# Autodesk Inventor assembly: EXCISS
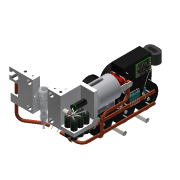
[picture p0: Inventor's stored thumbnail of the model, 180x180]
Saved by Autodesk Inventor 2017 (Build 210142000, 142)
## iProperties
Part Number: EXCISS
Material: Generisch
Document SubType Name: Assembly
Designer: Philomena-Theresa
Author: Philomena-Theresa
## Documents named in this file (28)
- C:\Seafile\Meine Bibliothek\Inventor\EXCISS\2019\HVU\HVU.iam
- C:\Seafile\Meine Bibliothek\Inventor\EXCISS\2019\HVU\HVU_sample_chamber_mount_plus.ipt
- C:\Seafile\Meine Bibliothek\Inventor\EXCISS\2019\HVU\HVU_PTFE_sleeve.ipt
- C:\Seafile\Meine Bibliothek\Inventor\EXCISS\2019\HVU\HVU_1N4007.ipt
- C:\Seafile\Meine Bibliothek\Inventor\EXCISS\2019\HVU\HVU_thyristor(TN2540-800G-TR).ipt
- C:\Seafile\Meine Bibliothek\Inventor\EXCISS\2019\HVU\HVU_ignition_coil.ipt
- C:\Seafile\Meine Bibliothek\Inventor\EXCISS\2019\HVU\HVU_DC_DC_converter_(M1730CQEA06065).ipt
- C:\Seafile\Meine Bibliothek\Inventor\EXCISS\2019\HVU\HVU_capacitor_MKP4_0,1µF_(450377).ipt
- C:\Seafile\Meine Bibliothek\Inventor\EXCISS\2019\HVU\HVU_capacitor_150µF_(LGN2X151MELB50).ipt
- C:\Seafile\Meine Bibliothek\Inventor\EXCISS\2019\HVU\HVU_resistor_WHS7_68R.ipt
- C:\Seafile\Meine Bibliothek\Inventor\EXCISS\2019\HVU\HVU_schunt.ipt
- C:\Seafile\Meine Bibliothek\Inventor\EXCISS\2019\HVU\HVU_PCB_trigger.ipt
- C:\Seafile\Meine Bibliothek\Inventor\EXCISS\2019\HVU\HVU_PCB_power_switch.ipt
- C:\Seafile\Meine Bibliothek\Inventor\EXCISS\2019\HVU\HVU_ferrit_cable_core_(28B0773-050).ipt
- C:\Seafile\Meine Bibliothek\Inventor\EXCISS\2019\HVU\HVU_sample_chamber_mount_minus.ipt
- C:\Seafile\Meine Bibliothek\Inventor\EXCISS\2019\HVU\HVU_sample_chamber.iam
- C:\Seafile\Meine Bibliothek\Inventor\EXCISS\2019\HVU\HVU_resistor_1M5_(VR25000001504JA100).ipt
- C:\Seafile\Meine Bibliothek\Inventor\EXCISS\2019\HVU\HVU_resistor_5M1_(VR25000005104JA100).ipt
- C:\Seafile\Meine Bibliothek\Inventor\EXCISS\2019\HVU\HVU_resistor_2M2_(VR25000002204JA100).ipt
- C:\Seafile\Meine Bibliothek\Inventor\EXCISS\2019\HVU\HVU_wires_Darc.ipt
- C:\Seafile\Meine Bibliothek\Inventor\EXCISS\2019\HVU\HVU_ignition_coil_stud.ipt
- C:\Seafile\Meine Bibliothek\Inventor\EXCISS\2019\HVU\HVU_wires_Carc.ipt
- C:\Seafile\Meine Bibliothek\Inventor\EXCISS\2019\HVU\HVU_wires_resistor_WHS7.ipt
- C:\Seafile\Meine Bibliothek\Inventor\EXCISS\2019\HVU\HVU_wires_resistor.ipt
- C:\Seafile\Meine Bibliothek\Inventor\EXCISS\2019\HVU\HVU_wires_diodes.ipt
- C:\Seafile\Meine Bibliothek\Inventor\EXCISS\2019\HVU\HVU_diode_(BY16).ipt
- C:\Seafile\Meine Bibliothek\Inventor\EXCISS\2019\HVU\HVU_DIN_934_M3x0,5.ipt
- C:\Seafile\Meine Bibliothek\Inventor\EXCISS\2019\HVU\HVU_standoff_(DA_40MM).ipt
## Components (49 placed, 27 different names)
1. HVU_sample_chamber_mount_plus:1 — Passend:28, Fluchtend:6, Passend:47, Fluchtend:13, Passend:48, Passend:49, Passend:50, Passend:51, Passend:53, Passend:54, Passend:58, Winkel:3, Fluchtend:25, Passend:94, Fluchtend:27, Passend:102, Passend:103, Passend:104, Fluchtend:36, Fluchtend:39, Passend:117, Passend:118, Fluchtend:46, Fluchtend:52, Passend:147, Passend:152, Winkel:12, Winkel:13
2. HVU_PTFE_sleeve:1 — Passend:28, Fluchtend:6, Passend:92
3. HVU_1N4007:1 — Passend:34, Passend:36, Passend:171, Passend:173, Fluchtend:89, Fluchtend:90
4. HVU_thyristor(TN2540-800G-TR):1 — Passend:34, Passend:36, Passend:37, Winkel:2, Passend:39, Fluchtend:9, Fluchtend:79, Passend:171
5. HVU_ignition_coil:1 — Passend:37, Winkel:2, Passend:58, Winkel:3, Passend:123, Fluchtend:50, Fluchtend:51, Fluchtend:80, Passend:169, Fluchtend:88
6. HVU_DC_DC_converter_(M1730CQEA06065):1 — Passend:79, Fluchtend:43, Passend:149, Winkel:11, Passend:160, Passend:161, Passend:162, Passend:163, Passend:164, Passend:165, Fluchtend:91, Fluchtend:92, Fluchtend:93, Fluchtend:95, Fluchtend:96, Passend:175, Passend:176, Passend:177
7. HVU_capacitor_MKP4_0,1µF_(450377):1 — Passend:39, Fluchtend:9, Passend:56, Fluchtend:22, Passend:161, Passend:167, Passend:168, Fluchtend:78, Fluchtend:79, Fluchtend:80, Passend:169, Fluchtend:81, Passend:170, Fluchtend:83, Fluchtend:85, Passend:174
8. HVU_resistor_2M2_(VR25000002204JA100):1 — Passend:167, Passend:168, Fluchtend:78, Passend:172, Fluchtend:86, Fluchtend:87
9. HVU_diode_(BY16):1 — Passend:47, Fluchtend:13, Passend:101, Fluchtend:34, Fluchtend:35, Passend:123
10. HVU_diode_(BY16):2 — Passend:49, Passend:78, Fluchtend:27, Fluchtend:28, Fluchtend:29, Fluchtend:30, Fluchtend:31, Fluchtend:32, Passend:95, Passend:100
11. HVU_diode_(BY16):3 — Passend:48, Fluchtend:28, Passend:95
12. HVU_diode_(BY16):4 — Passend:53, Passend:77, Fluchtend:31, Passend:96, Passend:98, Passend:111, Fluchtend:45
13. HVU_diode_(BY16):5 — Passend:54, Fluchtend:32, Passend:96, Fluchtend:33, Passend:112
14. HVU_diode_(BY16):6 — Passend:51, Passend:77, Passend:78, Fluchtend:30, Passend:97, Passend:99
15. HVU_diode_(BY16):7 — Passend:50, Fluchtend:29, Passend:97
16. HVU_1N4007:2 — Passend:56, Fluchtend:22, Passend:170, Fluchtend:82, Fluchtend:84
17. HVU_resistor_5M1_(VR25000005104JA100):1 — Passend:155, Fluchtend:66, Passend:158, Fluchtend:72
18. HVU_1N4007:3 — Passend:144, Passend:145, Passend:152, Passend:166, Fluchtend:74, Fluchtend:75, Fluchtend:77
19. HVU_thyristor(TN2540-800G-TR):2 — Passend:144, Passend:145, Passend:150, Passend:151, Passend:153, Passend:166, Fluchtend:76
20. HVU_resistor_WHS7_68R:2 — Passend:72, Fluchtend:58, Passend:147, Passend:148, Passend:149
21. HVU_resistor_WHS7_68R:3 — Passend:72, Fluchtend:53, Fluchtend:58, Passend:148, Passend:150, Passend:153, Fluchtend:61, Fluchtend:62, Fluchtend:63, Fluchtend:64, Fluchtend:65
22. HVU_schunt:1 — Fluchtend:47, Passend:137, Passend:138, Passend:139
23. HVU_PCB_trigger:1 — Passend:79, Winkel:11, Passend:164, Fluchtend:99
24. HVU_PCB_power_switch:1 — Passend:177, Fluchtend:100, Passend:178
25. HVU_ferrit_cable_core_(28B0773-050):1 — Passend:175, Passend:176, Fluchtend:99, Fluchtend:100, Passend:178
26. HVU_sample_chamber_mount_minus:1 — Passend:93, Fluchtend:25, Passend:94, Winkel:7, Passend:113, Passend:114, Fluchtend:48, Fluchtend:49
27. HVU_sample_chamber:1 [sub-assembly] — Passend:92, Passend:93, Winkel:7
28. HVU_ignition_coil_stud:1 — Passend:103, Fluchtend:37
29. HVU_ignition_coil_stud:2 — Passend:102, Fluchtend:36, Fluchtend:37, Fluchtend:38
30. HVU_ignition_coil_stud:3 — Passend:104, Fluchtend:38
31. HVU_wires_Carc:1 — Fluchtend:40, Passend:105, Passend:106, Passend:107, Passend:108, Passend:109, Passend:110, Passend:111, Passend:112, Passend:132, Passend:133, Winkel:9, Fluchtend:48, Fluchtend:49, Fluchtend:50, Fluchtend:51, Fluchtend:52
32. HVU_wires_Darc:1 — Fluchtend:33, Passend:98, Passend:99, Passend:100, Passend:101, Fluchtend:34, Fluchtend:35, Fluchtend:45, Passend:132, Passend:133
33. HVU_wires_resistor_WHS7:1 — Fluchtend:60, Fluchtend:61, Fluchtend:62, Fluchtend:63, Fluchtend:64, Fluchtend:65
34. HVU_wires_resistor:1 — Fluchtend:68, Fluchtend:69, Fluchtend:70, Fluchtend:71, Fluchtend:72, Fluchtend:73, Passend:172, Fluchtend:85, Fluchtend:86, Fluchtend:87, Fluchtend:91, Fluchtend:94, Fluchtend:95, Fluchtend:96, Fluchtend:97, Fluchtend:98
35. HVU_wires_diodes:1 — Fluchtend:75, Fluchtend:76, Fluchtend:77, Fluchtend:81, Fluchtend:82, Fluchtend:83, Fluchtend:84, Passend:173, Fluchtend:88, Fluchtend:89, Fluchtend:90
36. HVU_resistor_1M5_(VR25000001504JA100):7 — Fluchtend:92, Fluchtend:93, Fluchtend:94, Passend:174, Fluchtend:97, Fluchtend:98
37. DIN 934 - ersetzt durch DIN EN 24032/28673/28674 M3:3 — Passend:181, Winkel:14
38. DIN 934 - ersetzt durch DIN EN 24032/28673/28674 M3:4 — Passend:182, Winkel:14
39. HVU_resistor_1M5_(VR25000001504JA100):1 — Passend:155, Fluchtend:66, Passend:158, Passend:162, Fluchtend:67, Fluchtend:69, Passend:165, Fluchtend:71
40. HVU_resistor_1M5_(VR25000001504JA100):2 — Fluchtend:70
41. HVU_resistor_1M5_(VR25000001504JA100):3
42. HVU_resistor_1M5_(VR25000001504JA100):4
43. HVU_resistor_1M5_(VR25000001504JA100):5
44. HVU_resistor_1M5_(VR25000001504JA100):6 — Passend:163, Fluchtend:73
45. HVU_capacitor_150µF_(LGN2X151MELB50):1 — Passend:107, Passend:110, Passend:126, Passend:179, Fluchtend:101
46. HVU_capacitor_150µF_(LGN2X151MELB50):2 — Passend:106, Passend:109, Passend:180
47. HVU_capacitor_150µF_(LGN2X151MELB50):3 — Passend:105, Passend:108, Passend:124, Passend:125, Passend:139, Winkel:12
48. HVU_standoff_(DA_40MM):1 — Passend:179, Passend:180, Winkel:13, Fluchtend:101, Passend:181
49. HVU_standoff_(DA_40MM):2 — Passend:182
## Component patterns: (6 elements, first: HVU_resistor_1M5_(VR25000001504JA100):1), (3 elements, first: HVU_capacitor_150µF_(LGN2X151MELB50):1), (2 elements, first: HVU_standoff_(DA_40MM):1)
## Relationships (183: Mate 98, Flush 75, Angle 9, Symmetry 1)
- Passend:28 [Mate]: HVU_sample_chamber_mount_plus:1 ↔ HVU_PTFE_sleeve:1
- Fluchtend:6 [Flush] (-5.67 mm): HVU_sample_chamber_mount_plus:1 ↔ HVU_PTFE_sleeve:1
- Passend:34 [Mate] (0.39 mm): HVU_1N4007:1 ↔ HVU_thyristor(TN2540-800G-TR):1
- Passend:36 [Mate]: HVU_1N4007:1 ↔ HVU_thyristor(TN2540-800G-TR):1
- Passend:37 [Mate]: HVU_thyristor(TN2540-800G-TR):1 ↔ HVU_ignition_coil:1
- Winkel:2 [Angle] (0 deg): HVU_thyristor(TN2540-800G-TR):1 ↔ HVU_ignition_coil:1
- Passend:39 [Mate]: HVU_thyristor(TN2540-800G-TR):1 ↔ HVU_capacitor_MKP4_0,1µF_(450377):1
- Fluchtend:9 [Flush]: HVU_thyristor(TN2540-800G-TR):1 ↔ HVU_capacitor_MKP4_0,1µF_(450377):1
- Passend:47 [Mate]: HVU_sample_chamber_mount_plus:1 ↔ HVU_diode_(BY16):1
- Fluchtend:13 [Flush] (-1 mm): HVU_sample_chamber_mount_plus:1 ↔ HVU_diode_(BY16):1
- Passend:48 [Mate]: HVU_sample_chamber_mount_plus:1 ↔ HVU_diode_(BY16):3
- Passend:49 [Mate]: HVU_sample_chamber_mount_plus:1 ↔ HVU_diode_(BY16):2
- Passend:50 [Mate]: HVU_sample_chamber_mount_plus:1 ↔ HVU_diode_(BY16):7
- Passend:51 [Mate]: HVU_sample_chamber_mount_plus:1 ↔ HVU_diode_(BY16):6
- Passend:53 [Mate]: HVU_sample_chamber_mount_plus:1 ↔ HVU_diode_(BY16):4
- Passend:54 [Mate]: HVU_sample_chamber_mount_plus:1 ↔ HVU_diode_(BY16):5
- Passend:56 [Mate] (1.5 mm): HVU_capacitor_MKP4_0,1µF_(450377):1 ↔ HVU_1N4007:2
- Fluchtend:22 [Flush]: HVU_capacitor_MKP4_0,1µF_(450377):1 ↔ HVU_1N4007:2
- Passend:58 [Mate] (3 mm): HVU_sample_chamber_mount_plus:1 ↔ HVU_ignition_coil:1
- Winkel:3 [Angle] (270 deg): HVU_sample_chamber_mount_plus:1 ↔ HVU_ignition_coil:1
- Passend:72 [Mate] (9 mm): HVU_resistor_WHS7_68R:2 ↔ HVU_resistor_WHS7_68R:3
- Passend:77 [Mate]: HVU_diode_(BY16):4 ↔ HVU_diode_(BY16):6
- Passend:78 [Mate]: HVU_diode_(BY16):2 ↔ HVU_diode_(BY16):6
- Passend:79 [Mate] (1 mm): HVU_DC_DC_converter_(M1730CQEA06065):1 ↔ HVU_PCB_trigger:1
- Passend:92 [Mate]: HVU_PTFE_sleeve:1 ↔ HVU_sample_chamber:1
- Passend:93 [Mate]: HVU_sample_chamber_mount_minus:1 ↔ HVU_sample_chamber:1
- Fluchtend:25 [Flush]: HVU_sample_chamber_mount_plus:1 ↔ HVU_sample_chamber_mount_minus:1
- Passend:94 [Mate] (30 mm): HVU_sample_chamber_mount_plus:1 ↔ HVU_sample_chamber_mount_minus:1
- Winkel:7 [Angle] (0 deg): HVU_sample_chamber_mount_minus:1 ↔ HVU_sample_chamber:1
- Fluchtend:27 [Flush] (6 mm): HVU_sample_chamber_mount_plus:1 ↔ HVU_diode_(BY16):2
- Fluchtend:28 [Flush]: HVU_diode_(BY16):2 ↔ HVU_diode_(BY16):3
- Fluchtend:29 [Flush]: HVU_diode_(BY16):2 ↔ HVU_diode_(BY16):7
- Fluchtend:30 [Flush]: HVU_diode_(BY16):2 ↔ HVU_diode_(BY16):6
- Fluchtend:31 [Flush]: HVU_diode_(BY16):2 ↔ HVU_diode_(BY16):4
- Fluchtend:32 [Flush]: HVU_diode_(BY16):2 ↔ HVU_diode_(BY16):5
- Passend:95 [Mate]: HVU_diode_(BY16):2 ↔ HVU_diode_(BY16):3
- Passend:96 [Mate]: HVU_diode_(BY16):4 ↔ HVU_diode_(BY16):5
- Passend:97 [Mate]: HVU_diode_(BY16):6 ↔ HVU_diode_(BY16):7
- Fluchtend:33 [Flush]: HVU_diode_(BY16):5 ↔ HVU_wires_Darc:1
- Passend:98 [Mate]: HVU_diode_(BY16):4 ↔ HVU_wires_Darc:1
- Passend:99 [Mate]: HVU_diode_(BY16):6 ↔ HVU_wires_Darc:1
- Passend:100 [Mate]: HVU_diode_(BY16):2 ↔ HVU_wires_Darc:1
- Passend:101 [Mate]: HVU_diode_(BY16):1 ↔ HVU_wires_Darc:1
- Fluchtend:34 [Flush]: HVU_diode_(BY16):1 ↔ HVU_wires_Darc:1
- Fluchtend:35 [Flush]: HVU_diode_(BY16):1 ↔ HVU_wires_Darc:1
- Passend:102 [Mate]: HVU_sample_chamber_mount_plus:1 ↔ HVU_ignition_coil_stud:2
- Passend:103 [Mate]: HVU_sample_chamber_mount_plus:1 ↔ HVU_ignition_coil_stud:1
- Passend:104 [Mate]: HVU_sample_chamber_mount_plus:1 ↔ HVU_ignition_coil_stud:3
- Fluchtend:36 [Flush]: HVU_sample_chamber_mount_plus:1 ↔ HVU_ignition_coil_stud:2
- Fluchtend:37 [Flush]: HVU_ignition_coil_stud:1 ↔ HVU_ignition_coil_stud:2
- Fluchtend:38 [Flush]: HVU_ignition_coil_stud:2 ↔ HVU_ignition_coil_stud:3
- Fluchtend:39 [Flush] (-9 mm): HVU_sample_chamber_mount_plus:1
- Fluchtend:40 [Flush]: HVU_wires_Carc:1
- Passend:105 [Mate]: HVU_wires_Carc:1 ↔ HVU_capacitor_150µF_(LGN2X151MELB50):3
- Passend:106 [Mate]: HVU_wires_Carc:1 ↔ HVU_capacitor_150µF_(LGN2X151MELB50):2
- Passend:107 [Mate]: HVU_wires_Carc:1 ↔ HVU_capacitor_150µF_(LGN2X151MELB50):1
- Passend:108 [Mate]: HVU_wires_Carc:1 ↔ HVU_capacitor_150µF_(LGN2X151MELB50):3
- Passend:109 [Mate]: HVU_wires_Carc:1 ↔ HVU_capacitor_150µF_(LGN2X151MELB50):2
- Passend:110 [Mate]: HVU_wires_Carc:1 ↔ HVU_capacitor_150µF_(LGN2X151MELB50):1
- Passend:111 [Mate]: HVU_diode_(BY16):4 ↔ HVU_wires_Carc:1
- Passend:112 [Mate]: HVU_diode_(BY16):5 ↔ HVU_wires_Carc:1
- Passend:113 [Mate]: HVU_sample_chamber_mount_minus:1
- Passend:114 [Mate]: HVU_sample_chamber_mount_minus:1
- Passend:115 [Mate]
- Passend:116 [Mate]
- Passend:117 [Mate]: HVU_sample_chamber_mount_plus:1
- Passend:118 [Mate]: HVU_sample_chamber_mount_plus:1
- Passend:119 [Mate]
- Passend:120 [Mate]
- Fluchtend:41 [Flush] (-5 mm)
- Fluchtend:42 [Flush] (-5 mm)
- Fluchtend:43 [Flush] (0.4 mm): HVU_DC_DC_converter_(M1730CQEA06065):1
- Passend:121 [Mate]
- Passend:122 [Mate]
- Fluchtend:44 [Flush] (-5 mm)
- Passend:123 [Mate]: HVU_ignition_coil:1 ↔ HVU_diode_(BY16):1
- Passend:124 [Mate] (2.125 mm): HVU_capacitor_150µF_(LGN2X151MELB50):3
- Passend:125 [Mate]: HVU_capacitor_150µF_(LGN2X151MELB50):3
- Passend:126 [Mate]: HVU_capacitor_150µF_(LGN2X151MELB50):1
- Passend:127 [Mate]
- Passend:128 [Mate]
- Passend:129 [Mate] (-15.5 mm)
- Fluchtend:45 [Flush]: HVU_diode_(BY16):4 ↔ HVU_wires_Darc:1
- Passend:132 [Mate]: HVU_wires_Carc:1 ↔ HVU_wires_Darc:1
- Passend:133 [Mate]: HVU_wires_Carc:1 ↔ HVU_wires_Darc:1
- Fluchtend:46 [Flush] (7 mm): HVU_sample_chamber_mount_plus:1
- Passend:134 [Mate]
- Passend:135 [Mate]
- Passend:136 [Mate]
- Winkel:8 [Angle] (45 deg)
- Fluchtend:47 [Flush] (0.5 mm): HVU_schunt:1
- Symmetrie:1
- Passend:137 [Mate]: HVU_schunt:1
- Winkel:9 [Angle] (90 deg): HVU_wires_Carc:1
- Passend:138 [Mate] (5.5 mm): HVU_schunt:1
- Passend:139 [Mate] (15.5 mm): HVU_schunt:1 ↔ HVU_capacitor_150µF_(LGN2X151MELB50):3
- Fluchtend:48 [Flush]: HVU_sample_chamber_mount_minus:1 ↔ HVU_wires_Carc:1
- Fluchtend:49 [Flush]: HVU_sample_chamber_mount_minus:1 ↔ HVU_wires_Carc:1
- Fluchtend:50 [Flush]: HVU_ignition_coil:1 ↔ HVU_wires_Carc:1
- Fluchtend:51 [Flush]: HVU_ignition_coil:1 ↔ HVU_wires_Carc:1
- Fluchtend:52 [Flush]: HVU_sample_chamber_mount_plus:1 ↔ HVU_wires_Carc:1
- Fluchtend:53 [Flush]: HVU_resistor_WHS7_68R:3
- Fluchtend:58 [Flush]: HVU_resistor_WHS7_68R:2 ↔ HVU_resistor_WHS7_68R:3
- Passend:144 [Mate] (0.39 mm): HVU_1N4007:3 ↔ HVU_thyristor(TN2540-800G-TR):2
- Passend:145 [Mate] (-1.2 mm): HVU_1N4007:3 ↔ HVU_thyristor(TN2540-800G-TR):2
- Passend:147 [Mate] (-4.6 mm): HVU_sample_chamber_mount_plus:1 ↔ HVU_resistor_WHS7_68R:2
- Passend:148 [Mate]: HVU_resistor_WHS7_68R:2 ↔ HVU_resistor_WHS7_68R:3
- Passend:149 [Mate] (-4.5 mm): HVU_DC_DC_converter_(M1730CQEA06065):1 ↔ HVU_resistor_WHS7_68R:2
- Passend:150 [Mate] (3 mm): HVU_thyristor(TN2540-800G-TR):2 ↔ HVU_resistor_WHS7_68R:3
- Passend:151 [Mate] (-1 mm): HVU_thyristor(TN2540-800G-TR):2
- Passend:152 [Mate] (35.5 mm): HVU_sample_chamber_mount_plus:1 ↔ HVU_1N4007:3
- Passend:153 [Mate] (-2 mm): HVU_thyristor(TN2540-800G-TR):2 ↔ HVU_resistor_WHS7_68R:3
- Fluchtend:60 [Flush]: HVU_wires_resistor_WHS7:1
- Fluchtend:61 [Flush]: HVU_resistor_WHS7_68R:3 ↔ HVU_wires_resistor_WHS7:1
- Fluchtend:62 [Flush]: HVU_resistor_WHS7_68R:3 ↔ HVU_wires_resistor_WHS7:1
- Fluchtend:63 [Flush]: HVU_resistor_WHS7_68R:3 ↔ HVU_wires_resistor_WHS7:1
- Fluchtend:64 [Flush]: HVU_resistor_WHS7_68R:3 ↔ HVU_wires_resistor_WHS7:1
- Fluchtend:65 [Flush]: HVU_resistor_WHS7_68R:3 ↔ HVU_wires_resistor_WHS7:1
- Passend:155 [Mate]: HVU_resistor_5M1_(VR25000005104JA100):1 ↔ HVU_resistor_1M5_(VR25000001504JA100):1
- Fluchtend:66 [Flush]: HVU_resistor_5M1_(VR25000005104JA100):1 ↔ HVU_resistor_1M5_(VR25000001504JA100):1
- Passend:158 [Mate] (8 mm): HVU_resistor_5M1_(VR25000005104JA100):1 ↔ HVU_resistor_1M5_(VR25000001504JA100):1
- Winkel:11 [Angle] (0 deg): HVU_DC_DC_converter_(M1730CQEA06065):1 ↔ HVU_PCB_trigger:1
- Passend:160 [Mate]: HVU_DC_DC_converter_(M1730CQEA06065):1
- Passend:161 [Mate] (1 mm): HVU_DC_DC_converter_(M1730CQEA06065):1 ↔ HVU_capacitor_MKP4_0,1µF_(450377):1
- Passend:162 [Mate] (-0.5 mm): HVU_DC_DC_converter_(M1730CQEA06065):1 ↔ HVU_resistor_1M5_(VR25000001504JA100):1
- Passend:163 [Mate] (4 mm): HVU_DC_DC_converter_(M1730CQEA06065):1 ↔ HVU_resistor_1M5_(VR25000001504JA100):6
- Passend:164 [Mate]: HVU_DC_DC_converter_(M1730CQEA06065):1 ↔ HVU_PCB_trigger:1
- Fluchtend:67 [Flush]: HVU_resistor_1M5_(VR25000001504JA100):1
- Fluchtend:68 [Flush]: HVU_wires_resistor:1
- Fluchtend:69 [Flush]: HVU_wires_resistor:1 ↔ HVU_resistor_1M5_(VR25000001504JA100):1
- Fluchtend:70 [Flush]: HVU_wires_resistor:1 ↔ HVU_resistor_1M5_(VR25000001504JA100):2
- Passend:165 [Mate] (2 mm): HVU_DC_DC_converter_(M1730CQEA06065):1 ↔ HVU_resistor_1M5_(VR25000001504JA100):1
- Fluchtend:71 [Flush]: HVU_wires_resistor:1 ↔ HVU_resistor_1M5_(VR25000001504JA100):1
- Fluchtend:72 [Flush]: HVU_resistor_5M1_(VR25000005104JA100):1 ↔ HVU_wires_resistor:1
- Fluchtend:73 [Flush]: HVU_wires_resistor:1 ↔ HVU_resistor_1M5_(VR25000001504JA100):6
- Passend:166 [Mate]: HVU_1N4007:3 ↔ HVU_thyristor(TN2540-800G-TR):2
- Fluchtend:74 [Flush]: HVU_1N4007:3
- Fluchtend:75 [Flush]: HVU_1N4007:3 ↔ HVU_wires_diodes:1
- Fluchtend:76 [Flush]: HVU_thyristor(TN2540-800G-TR):2 ↔ HVU_wires_diodes:1
- Winkel:12 [Angle] (90 deg): HVU_sample_chamber_mount_plus:1 ↔ HVU_capacitor_150µF_(LGN2X151MELB50):3
- Fluchtend:77 [Flush]: HVU_1N4007:3 ↔ HVU_wires_diodes:1
- Passend:167 [Mate] (1.35 mm): HVU_capacitor_MKP4_0,1µF_(450377):1 ↔ HVU_resistor_2M2_(VR25000002204JA100):1
- Passend:168 [Mate] (0.525 mm): HVU_capacitor_MKP4_0,1µF_(450377):1 ↔ HVU_resistor_2M2_(VR25000002204JA100):1
- Fluchtend:78 [Flush] (3 mm): HVU_capacitor_MKP4_0,1µF_(450377):1 ↔ HVU_resistor_2M2_(VR25000002204JA100):1
- Fluchtend:79 [Flush] (-0.65 mm): HVU_thyristor(TN2540-800G-TR):1 ↔ HVU_capacitor_MKP4_0,1µF_(450377):1
- Fluchtend:80 [Flush]: HVU_ignition_coil:1 ↔ HVU_capacitor_MKP4_0,1µF_(450377):1
- Passend:169 [Mate] (7.5 mm): HVU_ignition_coil:1 ↔ HVU_capacitor_MKP4_0,1µF_(450377):1
- Fluchtend:81 [Flush]: HVU_capacitor_MKP4_0,1µF_(450377):1 ↔ HVU_wires_diodes:1
- Passend:170 [Mate]: HVU_capacitor_MKP4_0,1µF_(450377):1 ↔ HVU_1N4007:2
- Fluchtend:82 [Flush]: HVU_1N4007:2 ↔ HVU_wires_diodes:1
- Fluchtend:83 [Flush]: HVU_capacitor_MKP4_0,1µF_(450377):1 ↔ HVU_wires_diodes:1
- Fluchtend:84 [Flush]: HVU_1N4007:2 ↔ HVU_wires_diodes:1
- Passend:171 [Mate] (-1.5 mm): HVU_1N4007:1 ↔ HVU_thyristor(TN2540-800G-TR):1
- Passend:172 [Mate]: HVU_resistor_2M2_(VR25000002204JA100):1 ↔ HVU_wires_resistor:1
- Fluchtend:85 [Flush]: HVU_capacitor_MKP4_0,1µF_(450377):1 ↔ HVU_wires_resistor:1
- Fluchtend:86 [Flush]: HVU_resistor_2M2_(VR25000002204JA100):1 ↔ HVU_wires_resistor:1
- Fluchtend:87 [Flush]: HVU_resistor_2M2_(VR25000002204JA100):1 ↔ HVU_wires_resistor:1
- Passend:173 [Mate]: HVU_1N4007:1 ↔ HVU_wires_diodes:1
- Fluchtend:88 [Flush]: HVU_ignition_coil:1 ↔ HVU_wires_diodes:1
- Fluchtend:89 [Flush]: HVU_1N4007:1 ↔ HVU_wires_diodes:1
- Fluchtend:90 [Flush]: HVU_1N4007:1 ↔ HVU_wires_diodes:1
- Fluchtend:91 [Flush]: HVU_DC_DC_converter_(M1730CQEA06065):1 ↔ HVU_wires_resistor:1
- Fluchtend:92 [Flush] (2 mm): HVU_DC_DC_converter_(M1730CQEA06065):1 ↔ HVU_resistor_1M5_(VR25000001504JA100):7
- Fluchtend:93 [Flush]: HVU_DC_DC_converter_(M1730CQEA06065):1 ↔ HVU_resistor_1M5_(VR25000001504JA100):7
- Fluchtend:94 [Flush]: HVU_wires_resistor:1 ↔ HVU_resistor_1M5_(VR25000001504JA100):7
- Fluchtend:95 [Flush]: HVU_DC_DC_converter_(M1730CQEA06065):1 ↔ HVU_wires_resistor:1
- Fluchtend:96 [Flush]: HVU_DC_DC_converter_(M1730CQEA06065):1 ↔ HVU_wires_resistor:1
- Passend:174 [Mate] (-0.675 mm): HVU_capacitor_MKP4_0,1µF_(450377):1 ↔ HVU_resistor_1M5_(VR25000001504JA100):7
- Fluchtend:97 [Flush]: HVU_wires_resistor:1 ↔ HVU_resistor_1M5_(VR25000001504JA100):7
- Fluchtend:98 [Flush]: HVU_wires_resistor:1 ↔ HVU_resistor_1M5_(VR25000001504JA100):7
- Passend:175 [Mate] (0.5 mm): HVU_DC_DC_converter_(M1730CQEA06065):1 ↔ HVU_ferrit_cable_core_(28B0773-050):1
- Passend:176 [Mate] (-1 mm): HVU_DC_DC_converter_(M1730CQEA06065):1 ↔ HVU_ferrit_cable_core_(28B0773-050):1
- Fluchtend:99 [Flush]: HVU_PCB_trigger:1 ↔ HVU_ferrit_cable_core_(28B0773-050):1
- Passend:177 [Mate] (1 mm): HVU_DC_DC_converter_(M1730CQEA06065):1 ↔ HVU_PCB_power_switch:1
- Fluchtend:100 [Flush]: HVU_PCB_power_switch:1 ↔ HVU_ferrit_cable_core_(28B0773-050):1
- Passend:178 [Mate] (6 mm): HVU_PCB_power_switch:1 ↔ HVU_ferrit_cable_core_(28B0773-050):1
- Passend:179 [Mate] (19.55 mm): HVU_capacitor_150µF_(LGN2X151MELB50):1 ↔ HVU_standoff_(DA_40MM):1
- Passend:180 [Mate] (20.532 mm): HVU_capacitor_150µF_(LGN2X151MELB50):2 ↔ HVU_standoff_(DA_40MM):1
- Winkel:13 [Angle] (0 deg): HVU_sample_chamber_mount_plus:1 ↔ HVU_standoff_(DA_40MM):1
- Fluchtend:101 [Flush] (-14.7 mm): HVU_capacitor_150µF_(LGN2X151MELB50):1 ↔ HVU_standoff_(DA_40MM):1
- Passend:181 [Mate]: DIN 934 - ersetzt durch DIN EN 24032/28673/28674 M3:3 ↔ HVU_standoff_(DA_40MM):1
- Passend:182 [Mate]: DIN 934 - ersetzt durch DIN EN 24032/28673/28674 M3:4 ↔ HVU_standoff_(DA_40MM):2
- Winkel:14 [Angle] (0 deg): DIN 934 - ersetzt durch DIN EN 24032/28673/28674 M3:3 ↔ DIN 934 - ersetzt durch DIN EN 24032/28673/28674 M3:4
